# Autodesk Inventor assembly: HBLTBBN45
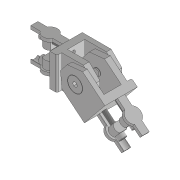
[picture p0: Inventor's stored thumbnail of the model, 180x180]
Saved by Autodesk Inventor 2020 (Build 240168000, 168)
## iProperties
Created: 2021-12-05
Part Number: HBLTBBN45
Document SubType Name: Assembly
Designer: ken113
Author: ken113
## Documents named in this file (2)
- D:\Document\Github\Eto_Project\Hardware\Parts\MISUMI\HBLTBBN45-SET_Autodesk_Inventor_2020_20211206\AIS2020\HBLTBBN45.iam
- D:\Document\Github\Eto_Project\Hardware\Parts\MISUMI\HBLTBBN45-SET_Autodesk_Inventor_2020_20211206\AIS2020\HBLTBBN45-SET.iam
## Components (2 placed, 1 different names)
1. HBLTBBN45-SET:1 [sub-assembly] — 挿入:1
2. HBLTBBN45-SET:2 [sub-assembly] — 挿入:1
## Relationships (1: Insert 1)
- 挿入:1 [Insert]: HBLTBBN45-SET:1 ↔ HBLTBBN45-SET:2
